# Autodesk Inventor assembly: Ankle_MIR
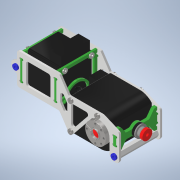
[picture p0: Inventor's stored thumbnail of the model, 180x180]
Saved by Autodesk Inventor 2020 (Build 240168000, 168)
## iProperties
Created: 2021-10-01
Part Number: Ankle_MIR
Document SubType Name: Assembly
Designer: Masato Kubotera
Author: Masato
## Documents named in this file (20)
- C:\Users\Masato\Desktop\OpenPlatform_ver3_0 - Ver4_1branch\LowerBody\Ankle\Ankle_MIR.iam
- C:\Users\Masato\Desktop\OpenPlatform_ver3_0 - Ver4_1branch\Ready_Made\B3M11xx.ipt
- C:\Users\Masato\Desktop\OpenPlatform_ver3_0 - Ver4_1branch\Ready_Made\B3M10xx.ipt
- C:\Users\Masato\Desktop\OpenPlatform_ver3_0 - Ver4_1branch\Ready_Made\SLSBF6-39_5-M3-N3.ipt
- C:\Users\Masato\Desktop\OpenPlatform_ver3_0 - Ver4_1branch\LowerBody\Ankle\Ankle_back_frame.ipt
- C:\Users\Masato\Desktop\OpenPlatform_ver3_0 - Ver4_1branch\LowerBody\Ankle\Ankle_front_frame.ipt
- C:\Users\Masato\Desktop\OpenPlatform_ver3_0 - Ver4_1branch\LowerBody\Ankle\Ankle_side_frame.ipt
- C:\Users\Masato\Desktop\OpenPlatform_ver3_0 - Ver4_1branch\Ready_Made\Screw\M2_6-15.ipt
- C:\Users\Masato\Desktop\OpenPlatform_ver3_0 - Ver4_1branch\Ready_Made\Screw\M2_6-20.ipt
- C:\Users\Masato\Desktop\OpenPlatform_ver3_0 - Ver4_1branch\Ready_Made\Screw\M3-6.ipt
- C:\Users\Masato\Desktop\OpenPlatform_ver3_0 - Ver4_1branch\Ready_Made\80F-0603.ipt
- C:\Users\Masato\Desktop\OpenPlatform_ver3_0 - Ver4_1branch\Ready_Made\FreeHorn.ipt
- C:\Users\Masato\Desktop\OpenPlatform_ver3_0 - Ver4_1branch\Ready_Made\CC-0612-15B.ipt
- C:\Users\Masato\Desktop\OpenPlatform_ver3_0 - Ver4_1branch\Ready_Made\Screw\FreeHorn_Screw.ipt
- C:\Users\Masato\Desktop\OpenPlatform_ver3_0 - Ver4_1branch\Ready_Made\S4-05-3W.ipt
- C:\Users\Masato\Desktop\OpenPlatform_ver3_0 - Ver4_1branch\Ready_Made\UUW-0412-10BH.ipt
- C:\Users\Masato\Desktop\OpenPlatform_ver3_0 - Ver4_1branch\Ready_Made\DBS4-6-4.ipt
- C:\Users\Masato\Desktop\OpenPlatform_ver3_0 - Ver4_1branch\Ready_Made\ClampHorn.ipt
- C:\Users\Masato\Desktop\OpenPlatform_ver3_0 - Ver4_1branch\Ready_Made\Screw\ClampHorn_Screw.ipt
- ClampHorn.ipt
## Components (36 placed, 18 different names)
1. B3M11xx:1 — フラッシュ:5, フラッシュ:4, 挿入:8, 挿入:7, 挿入:5, 挿入:4, 挿入:3, 挿入:1, 挿入:42, 挿入:53, 角度:5, 挿入:60, 挿入:62
2. B3M10xx:1 — 挿入:58, 挿入:18, 挿入:16, 挿入:17, 挿入:44, 挿入:43, 挿入:61, 挿入:63, 角度:5
3. SLSBF6-39_5-M3-N3:1 — 角度:2, 挿入:10, 挿入:9
4. SLSBF6-39_5-M3-N3:2 — 角度:3, 挿入:12, 挿入:11
5. Ankle_back_frame:1 — 挿入:58, 挿入:18, 挿入:16, 挿入:17, 角度:3, フラッシュ:3, メイト:7, メイト:6, 挿入:37, 挿入:38, 挿入:39, 挿入:59
6. Ankle_front_frame:1 — フラッシュ:1, メイト:5, メイト:4, 挿入:54, 角度:4, 挿入:55
7. Ankle_side_frame:1 — メイト:8, 挿入:8, 挿入:7, 挿入:5, 角度:2, 挿入:10, フラッシュ:3, メイト:7, メイト:6, フラッシュ:1, メイト:5, メイト:4, 挿入:12, 挿入:26, 挿入:25, 挿入:23, 挿入:31, 挿入:32
8. Ankle_side_frame:2 — 挿入:4, 挿入:3, 挿入:1, 挿入:9, 挿入:11, 挿入:27, 挿入:28, 挿入:30, 挿入:33, 挿入:34
9. M2_6-15:1 — 挿入:26
10. M2_6-15:2 — 挿入:25
11. M2_6-15:3 — 挿入:23
12. M2_6-20:1 — 挿入:27
13. M2_6-20:2 — 挿入:28
14. M2_6-20:3 — 挿入:30
15. M3-6:1 — 挿入:31
16. M3-6:2 — 挿入:32
17. M3-6:3 — 挿入:33
18. M3-6:4 — 挿入:34
19. M2_6-20:4 — 挿入:47
20. M2_6-15:4 — 挿入:37
21. M2_6-15:5 — 挿入:38
22. M2_6-15:6 — 挿入:39
23. M2_6-15:7 — 挿入:59
24. 80F-0603:1 — 挿入:52
25. FreeHorn:1 — 挿入:42
26. Ankle_back_frame:2 — 挿入:44, 挿入:43, 挿入:47, 挿入:48
27. M2_6-20:5 — 挿入:48
28. CC-0612-15B:1 — 挿入:52, 挿入:56
29. FreeHorn_Screw:1 — 挿入:53
30. S4-05-3W:1 — 挿入:54, 角度:4
31. UUW-0412-10BH:1 — 挿入:56, 挿入:55, 挿入:57
32. DBS4-6-4:1 — 挿入:57
33. ClampHorn:1 — 挿入:60, 角度:5
34. ClampHorn:2 — 挿入:61, 角度:5
35. ClampHorn_Screw:1 — 挿入:62
36. ClampHorn_Screw:2 — 挿入:63
## Relationships (57: Insert 43, Mate 6, Angle 5, Flush 3)
- フラッシュ:5 [Flush]: B3M11xx:1
- フラッシュ:4 [Mate]: B3M11xx:1
- 挿入:58 [Insert]: B3M10xx:1 ↔ Ankle_back_frame:1
- 挿入:18 [Insert]: B3M10xx:1 ↔ Ankle_back_frame:1
- 挿入:16 [Insert]: B3M10xx:1 ↔ Ankle_back_frame:1
- 挿入:17 [Insert]: B3M10xx:1 ↔ Ankle_back_frame:1
- 角度:3 [Angle] (0 deg): SLSBF6-39_5-M3-N3:2 ↔ Ankle_back_frame:1
- メイト:8 [Mate] (19.75 mm): Ankle_side_frame:1
- 挿入:8 [Insert]: B3M11xx:1 ↔ Ankle_side_frame:1
- 挿入:7 [Insert]: B3M11xx:1 ↔ Ankle_side_frame:1
- 挿入:5 [Insert]: B3M11xx:1 ↔ Ankle_side_frame:1
- 角度:2 [Angle] (0 deg): SLSBF6-39_5-M3-N3:1 ↔ Ankle_side_frame:1
- 挿入:10 [Insert]: SLSBF6-39_5-M3-N3:1 ↔ Ankle_side_frame:1
- フラッシュ:3 [Flush]: Ankle_back_frame:1 ↔ Ankle_side_frame:1
- メイト:7 [Mate] (0.01 mm): Ankle_back_frame:1 ↔ Ankle_side_frame:1
- メイト:6 [Mate] (0.01 mm): Ankle_back_frame:1 ↔ Ankle_side_frame:1
- フラッシュ:1 [Flush]: Ankle_front_frame:1 ↔ Ankle_side_frame:1
- メイト:5 [Mate] (0.01 mm): Ankle_front_frame:1 ↔ Ankle_side_frame:1
- メイト:4 [Mate] (0.01 mm): Ankle_front_frame:1 ↔ Ankle_side_frame:1
- 挿入:12 [Insert]: SLSBF6-39_5-M3-N3:2 ↔ Ankle_side_frame:1
- 挿入:4 [Insert]: B3M11xx:1 ↔ Ankle_side_frame:2
- 挿入:3 [Insert]: B3M11xx:1 ↔ Ankle_side_frame:2
- 挿入:1 [Insert]: B3M11xx:1 ↔ Ankle_side_frame:2
- 挿入:9 [Insert]: SLSBF6-39_5-M3-N3:1 ↔ Ankle_side_frame:2
- 挿入:11 [Insert]: SLSBF6-39_5-M3-N3:2 ↔ Ankle_side_frame:2
- 挿入:26 [Insert]: Ankle_side_frame:1 ↔ M2_6-15:1
- 挿入:25 [Insert]: Ankle_side_frame:1 ↔ M2_6-15:2
- 挿入:23 [Insert]: Ankle_side_frame:1 ↔ M2_6-15:3
- 挿入:27 [Insert]: Ankle_side_frame:2 ↔ M2_6-20:1
- 挿入:28 [Insert]: Ankle_side_frame:2 ↔ M2_6-20:2
- 挿入:30 [Insert]: Ankle_side_frame:2 ↔ M2_6-20:3
- 挿入:31 [Insert]: Ankle_side_frame:1 ↔ M3-6:1
- 挿入:32 [Insert]: Ankle_side_frame:1 ↔ M3-6:2
- 挿入:33 [Insert]: Ankle_side_frame:2 ↔ M3-6:3
- 挿入:34 [Insert]: Ankle_side_frame:2 ↔ M3-6:4
- 挿入:37 [Insert]: Ankle_back_frame:1 ↔ M2_6-15:4
- 挿入:38 [Insert]: Ankle_back_frame:1 ↔ M2_6-15:5
- 挿入:39 [Insert]: Ankle_back_frame:1 ↔ M2_6-15:6
- 挿入:59 [Insert]: Ankle_back_frame:1 ↔ M2_6-15:7
- 挿入:42 [Insert]: B3M11xx:1 ↔ FreeHorn:1
- 挿入:44 [Insert]: B3M10xx:1 ↔ Ankle_back_frame:2
- 挿入:43 [Insert]: B3M10xx:1 ↔ Ankle_back_frame:2
- 挿入:47 [Insert]: M2_6-20:4 ↔ Ankle_back_frame:2
- 挿入:48 [Insert]: Ankle_back_frame:2 ↔ M2_6-20:5
- 挿入:52 [Insert]: 80F-0603:1 ↔ CC-0612-15B:1
- 挿入:53 [Insert]: B3M11xx:1 ↔ FreeHorn_Screw:1
- 挿入:54 [Insert]: Ankle_front_frame:1 ↔ S4-05-3W:1
- 角度:4 [Angle] (0 deg): Ankle_front_frame:1 ↔ S4-05-3W:1
- 挿入:56 [Insert]: CC-0612-15B:1 ↔ UUW-0412-10BH:1
- 挿入:55 [Insert]: Ankle_front_frame:1 ↔ UUW-0412-10BH:1
- 挿入:57 [Insert]: UUW-0412-10BH:1 ↔ DBS4-6-4:1
- 角度:5 [Angle] (0 deg): B3M11xx:1 ↔ ClampHorn:1
- 挿入:60 [Insert]: B3M11xx:1 ↔ ClampHorn:1
- 挿入:61 [Insert]: B3M10xx:1 ↔ ClampHorn:2
- 挿入:62 [Insert]: B3M11xx:1 ↔ ClampHorn_Screw:1
- 挿入:63 [Insert]: B3M10xx:1 ↔ ClampHorn_Screw:2
- 角度:5 [Angle] (0 deg): B3M10xx:1 ↔ ClampHorn:2
